# Autodesk Inventor assembly: GFRP_T2_14
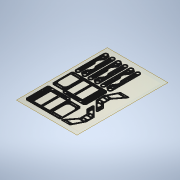
[picture p0: Inventor's stored thumbnail of the model, 180x180]
Saved by Autodesk Inventor 2020 (Build 240168000, 168)
## iProperties
Created: 2021-08-27
Part Number: GFRP_T2_14
Document SubType Name: Assembly
Designer: Masato
Author: Masato
## Documents named in this file (5)
- C:\Inventor\SUSTAINA-OP\Cam\GFRP_T2_14.iam
- C:\Inventor\SUSTAINA-OP\Cam\DisposableBoard.ipt
- C:\Inventor\SUSTAINA-OP\UpperBody\Trunk\Trunk_upper_side_frame.ipt
- C:\Inventor\SUSTAINA-OP\UpperBody\Head\Head_side_frame.ipt
- C:\Inventor\SUSTAINA-OP\LowerBody\Link\BackLink_frame.ipt
## Components (11 placed, 4 different names)
1. DisposableBoard:1 — メイト:2, メイト:1, フラッシュ:1, フラッシュ:2, メイト:4, メイト:5, フラッシュ:3, フラッシュ:4, メイト:7, メイト:9, メイト:12, メイト:13
2. Trunk_upper_side_frame:1 — メイト:4, フラッシュ:3, フラッシュ:4, メイト:6, フラッシュ:5, フラッシュ:6, メイト:8
3. Trunk_upper_side_frame:2 — メイト:5, メイト:6, フラッシュ:5, メイト:11, フラッシュ:7, 正接:1, 正接:2
4. Head_side_frame:1 — メイト:7, フラッシュ:6, メイト:8, メイト:10
5. Head_side_frame:2 — メイト:9, メイト:10, メイト:11
6. BackLink_frame:1 — メイト:12, フラッシュ:7, メイト:14, 正接:1
7. BackLink_frame:2 — メイト:13, メイト:14, 正接:2
8. BackLink_frame:3
9. BackLink_frame:4
10. BackLink_frame:5
11. BackLink_frame:6
## Component patterns: (3 elements, first: BackLink_frame:1 + BackLink_frame:2)
## Relationships (22: Mate 13, Flush 7, Tangent 2)
- メイト:2 [Mate]: DisposableBoard:1
- メイト:1 [Mate]: DisposableBoard:1
- フラッシュ:1 [Flush]: DisposableBoard:1
- フラッシュ:2 [Flush]: DisposableBoard:1
- メイト:4 [Mate]: DisposableBoard:1 ↔ Trunk_upper_side_frame:1
- メイト:5 [Mate]: DisposableBoard:1 ↔ Trunk_upper_side_frame:2
- フラッシュ:3 [Flush] (-2.5 mm): DisposableBoard:1 ↔ Trunk_upper_side_frame:1
- フラッシュ:4 [Flush] (2.5 mm): DisposableBoard:1 ↔ Trunk_upper_side_frame:1
- メイト:6 [Mate] (2.5 mm): Trunk_upper_side_frame:1 ↔ Trunk_upper_side_frame:2
- フラッシュ:5 [Flush]: Trunk_upper_side_frame:1 ↔ Trunk_upper_side_frame:2
- メイト:7 [Mate]: DisposableBoard:1 ↔ Head_side_frame:1
- フラッシュ:6 [Flush]: Trunk_upper_side_frame:1 ↔ Head_side_frame:1
- メイト:8 [Mate] (2.5 mm): Trunk_upper_side_frame:1 ↔ Head_side_frame:1
- メイト:9 [Mate]: DisposableBoard:1 ↔ Head_side_frame:2
- メイト:10 [Mate] (2.5 mm): Head_side_frame:1 ↔ Head_side_frame:2
- メイト:11 [Mate] (2.5 mm): Trunk_upper_side_frame:2 ↔ Head_side_frame:2
- メイト:12 [Mate]: DisposableBoard:1 ↔ BackLink_frame:1
- フラッシュ:7 [Flush]: Trunk_upper_side_frame:2 ↔ BackLink_frame:1
- メイト:13 [Mate]: DisposableBoard:1 ↔ BackLink_frame:2
- メイト:14 [Mate] (2.5 mm): BackLink_frame:1 ↔ BackLink_frame:2
- 正接:1 [Tangent] (2.5 mm): Trunk_upper_side_frame:2 ↔ BackLink_frame:1
- 正接:2 [Tangent] (2.5 mm): Trunk_upper_side_frame:2 ↔ BackLink_frame:2
